# Autodesk Inventor assembly: Pully 20mmx12mm
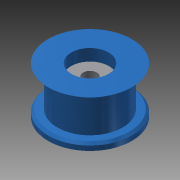
[picture p0: Inventor's stored thumbnail of the model, 180x180]
Saved by Autodesk Inventor 2013 (Build 170138000, 138)
## iProperties
Created: 2017-01-25
Part Number: Pully 20mmx12mm
Document SubType Name: Assembly
Designer: Herman de Vries
Author: Herman de Vries
## Documents named in this file (3)
- D:\Projects\Inventor\PaintBoid\Pully 20mmx12mm.iam
- D:\Projects\Inventor\PaintBoid\pully10mmx20mmx12mm.ipt
- D:\Projects\Inventor\PaintBoid\bearing 3mmx8mmx5mm.ipt
## Components (2 placed, 2 different names)
1. bearing 3mmx8mmx5mm:1 — Insert:1
2. pully10mmx20mmx12mm:1 — Insert:1
## Relationships (1: Insert 1)
- Insert:1 (-2.5 mm): bearing 3mmx8mmx5mm:1 ↔ pully10mmx20mmx12mm:1
